# Autodesk Inventor assembly: Tape Measure Scaler Assembly
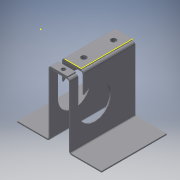
[picture p0: Inventor's stored thumbnail of the model, 180x180]
Saved by Autodesk Inventor 2016 (Build 200138000, 138)
## iProperties
Created: 2016-02-03
Part Number: Tape Measure Scaler Assembly
Document SubType Name: Assembly
Designer: GEH-Magnet School 1
Author: GEH-Magnet School 1
## Documents named in this file (3)
- C:\Users\GEH-Magnet School 1\Documents\Tape Measure Scaler Assembly.iam
- C:\Users\GEH-Magnet School 1\Documents\GitHub\2016RobotCADFiles\2x1\Tape Measure Dispenser Part 2.ipt
- C:\Users\GEH-Magnet School 1\Documents\GitHub\2016RobotCADFiles\2x1\Tape Measure Dispenser Side 1.ipt
## Components (2 placed, 2 different names)
1. Tape Measure Dispenser Part 2:1 — Flush:1, Mate:1, Mate:2
2. Tape Measure Dispenser Side 1:1 — Flush:1, Mate:1, Mate:2
## Relationships (3: Mate 2, Flush 1)
- Flush:1: Tape Measure Dispenser Part 2:1 ↔ Tape Measure Dispenser Side 1:1
- Mate:1: Tape Measure Dispenser Part 2:1 ↔ Tape Measure Dispenser Side 1:1
- Mate:2 (3.302 mm): Tape Measure Dispenser Part 2:1 ↔ Tape Measure Dispenser Side 1:1
